# Autodesk Inventor assembly: center-machine-assembly
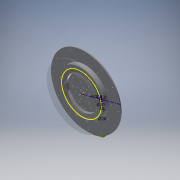
[picture p0: Inventor's stored thumbnail of the model, 180x180]
Saved by Autodesk Inventor 2018 (Build 220112000, 112)
## iProperties
Created: 2025-02-24
Part Number: center-machine-assembly
Document SubType Name: Assembly
Designer: neo
Author: neo
## Documents named in this file (8)
- C:\Users\neo\Documents\projects\kreion\design1\center-machine-assembly.iam
- C:\Users\neo\Documents\projects\kreion\design1\bearing100-80-10.ipt
- C:\Users\neo\Documents\projects\kreion\design1\bearing-base-lower-case.ipt
- C:\Users\neo\Documents\projects\kreion\design1\bearing-base-uppercase.ipt
- C:\Users\neo\Documents\projects\kreion\design1\piston-star-connector.ipt
- C:\Users\neo\Documents\projects\kreion\design1\rotor-case.ipt
- C:\Users\neo\Documents\projects\kreion\design1\piston-mount.ipt
- C:\Users\neo\Documents\projects\kreion\design1\piston.ipt
## Components (7 placed, 7 different names)
1. bearing100-80-10:1 — Tangent:1, Mate:1, Tangent:2, Mate:2, Mate:3, Tangent:4
2. bearing-base-lower-case:1 — Tangent:1, Mate:1, Tangent:3
3. bearing-base-uppercase:1 — Tangent:2, Mate:2, Tangent:3, Mate:5
4. piston-star-connector:1
5. rotor-case:1 — Mate:3, Tangent:4, Mate:4, Tangent:5, Tangent:6, Mate:6
6. piston-mount:1 — Mate:4, Tangent:5, Tangent:6
7. piston:1
## Relationships (12: Tangent 6, Mate 6)
- Tangent:1: bearing100-80-10:1 ↔ bearing-base-lower-case:1
- Mate:1: bearing100-80-10:1 ↔ bearing-base-lower-case:1
- Tangent:2: bearing100-80-10:1 ↔ bearing-base-uppercase:1
- Mate:2: bearing100-80-10:1 ↔ bearing-base-uppercase:1
- Tangent:3: bearing-base-lower-case:1 ↔ bearing-base-uppercase:1
- Mate:3: bearing100-80-10:1 ↔ rotor-case:1
- Tangent:4: bearing100-80-10:1 ↔ rotor-case:1
- Mate:4: rotor-case:1 ↔ piston-mount:1
- Tangent:5: rotor-case:1 ↔ piston-mount:1
- Tangent:6: rotor-case:1 ↔ piston-mount:1
- Mate:5: bearing-base-uppercase:1
- Mate:6: rotor-case:1
